# Autodesk Inventor assembly: base
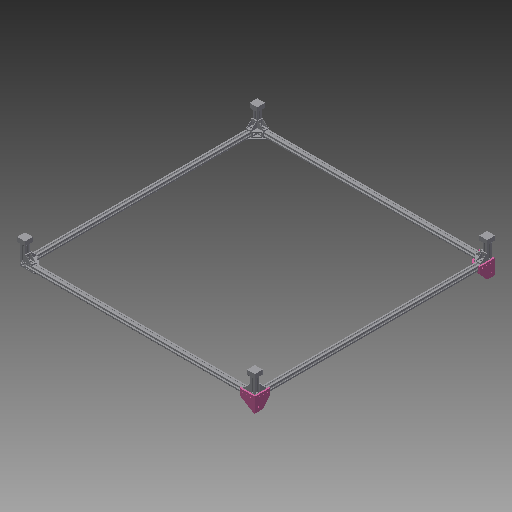
[picture p0: Inventor's stored thumbnail of the model, 512x512]
Saved by Autodesk Inventor 2019 (Build 230136000, 136)
## iProperties
Created: 2019-04-21
Part Number: base
Document SubType Name: Assembly
Designer: Alex Jones
Author: Alex Jones
## Documents named in this file (9)
- C:\Users\Alex Jones\Documents\Inventor\CNC\base.iam
- C:\Users\Alex Jones\Documents\Inventor\CNC\2020-1m.ipt
- C:\Users\Alex Jones\Documents\Inventor\CNC\2020-90.ipt
- C:\Users\Alex Jones\Documents\Inventor\CNC\2020-90-plate.ipt
- C:\Users\Alex Jones\Documents\Inventor\CNC\2020-3in.ipt
- C:\Users\Alex Jones\Documents\Inventor\CNC\baseFoot.ipt
- C:\Users\Alex Jones\Documents\Inventor\CNC\2020-950mm.ipt
- C:\Users\Alex Jones\Documents\Inventor\CNC\xIdler.ipt
- C:\Users\Alex Jones\Documents\Inventor\CNC\xIdlerMirror.ipt
## Components (28 placed, 8 different names)
1. 2020-950mm:1 — Mate:1, Flush:1, Flush:2, Flush:4, Mate:3, Flush:5, Flush:6, Flush:7, Flush:8, Flush:18, Mate:13, Mate:16, Flush:26, Mate:17, Flush:27, Mate:18, Flush:29, Mate:22, Mate:50
2. 2020-90:1 — Mate:1, Flush:1, Flush:2, Mate:2, Flush:3
3. 2020-1m:2 — Mate:4, Flush:7, Flush:8, Mate:5, Flush:10, Flush:12, Mate:12, Flush:19, Flush:20, Flush:21, Mate:14, Flush:28, Flush:30, Mate:21, Flush:35, Mate:31
4. 2020-1m:3 — Mate:2, Flush:3, Flush:4, Mate:6, Flush:9, Mate:9, Flush:23, Mate:15, Flush:25, Mate:24, Flush:32, Mate:45, Mate:46, Mate:47, Mate:49, Mate:51
5. 2020-950mm:2 — Mate:7, Flush:11, Mate:8, Mate:9, Flush:12, Flush:17, Flush:22, Flush:24, Flush:33, Mate:27, Mate:28, Flush:34, Mate:48
6. 2020-90:2 — Mate:6, Flush:9, Mate:8
7. 2020-90:3 — Mate:3, Flush:5, Flush:6, Mate:4
8. 2020-90:4 — Mate:5, Flush:10, Mate:7, Flush:11
9. 2020-90-plate:1 — Flush:18, Flush:19, Mate:13
10. 2020-90-plate:2 — Mate:12, Flush:17, Flush:20
11. 2020-3in:1 — Flush:21, Flush:22, Mate:14, Mate:29, Mate:30, Mate:35, Mate:36, Mate:37
12. 2020-3in:2 — Mate:17, Flush:27, Flush:28, Mate:19, Mate:20, Mate:38, Mate:39, Mate:40
13. 2020-3in:3 — Mate:16, Flush:25, Flush:26, Flush:31, Mate:23, Mate:25, Mate:41, Mate:42, Mate:43
14. 2020-3in:4 — Flush:23, Flush:24, Mate:15, Mate:26, Mate:32, Mate:33, Mate:34, Mate:44, Flush:36
15. 2020-90:5 — Mate:18, Flush:29, Mate:19
16. 2020-90:6 — Mate:20, Flush:30, Mate:21
17. 2020-90:7 — Mate:22, Flush:31, Mate:23
18. 2020-90:8 — Mate:24, Flush:32, Mate:25
19. 2020-90:9 — Flush:33, Mate:26, Mate:27
20. 2020-90:10 — Mate:28, Flush:34, Mate:29
21. 2020-90:11 — Flush:35, Mate:30, Mate:31
22. baseFoot:1 — Mate:32, Mate:33, Mate:34
23. baseFoot:2 — Mate:35, Mate:36, Mate:37
24. baseFoot:3 — Mate:38, Mate:39, Mate:40
25. baseFoot:4 — Mate:41, Mate:42, Mate:43
26. 2020-90:12 — Mate:44, Flush:36, Mate:45
27. xIdler:1 — Mate:46, Mate:47, Mate:48
28. xIdlerMirror:1 — Mate:49, Mate:50, Mate:51
## Relationships (81: Mate 49, Flush 32)
- Mate:1: 2020-950mm:1 ↔ 2020-90:1
- Flush:1: 2020-950mm:1 ↔ 2020-90:1
- Flush:2: 2020-950mm:1 ↔ 2020-90:1
- Mate:2: 2020-90:1 ↔ 2020-1m:3
- Flush:3: 2020-90:1 ↔ 2020-1m:3
- Flush:4: 2020-950mm:1 ↔ 2020-1m:3
- Mate:3: 2020-950mm:1 ↔ 2020-90:3
- Flush:5: 2020-950mm:1 ↔ 2020-90:3
- Flush:6: 2020-950mm:1 ↔ 2020-90:3
- Mate:4: 2020-1m:2 ↔ 2020-90:3
- Flush:7: 2020-950mm:1 ↔ 2020-1m:2
- Flush:8: 2020-950mm:1 ↔ 2020-1m:2
- Mate:5: 2020-1m:2 ↔ 2020-90:4
- Mate:6: 2020-1m:3 ↔ 2020-90:2
- Flush:9: 2020-1m:3 ↔ 2020-90:2
- Flush:10: 2020-1m:2 ↔ 2020-90:4
- Mate:7: 2020-950mm:2 ↔ 2020-90:4
- Flush:11: 2020-950mm:2 ↔ 2020-90:4
- Mate:8: 2020-950mm:2 ↔ 2020-90:2
- Mate:9: 2020-1m:3 ↔ 2020-950mm:2
- Flush:12: 2020-1m:2 ↔ 2020-950mm:2
- Mate:12: 2020-1m:2 ↔ 2020-90-plate:2
- Flush:17: 2020-950mm:2 ↔ 2020-90-plate:2
- Flush:18: 2020-950mm:1 ↔ 2020-90-plate:1
- Flush:19: 2020-1m:2 ↔ 2020-90-plate:1
- Mate:13: 2020-950mm:1 ↔ 2020-90-plate:1
- Flush:20: 2020-1m:2 ↔ 2020-90-plate:2
- Flush:21: 2020-1m:2 ↔ 2020-3in:1
- Flush:22: 2020-950mm:2 ↔ 2020-3in:1
- Mate:14: 2020-1m:2 ↔ 2020-3in:1
- Flush:23: 2020-1m:3 ↔ 2020-3in:4
- Flush:24: 2020-950mm:2 ↔ 2020-3in:4
- Mate:15: 2020-1m:3 ↔ 2020-3in:4
- Mate:16: 2020-950mm:1 ↔ 2020-3in:3
- Flush:25: 2020-1m:3 ↔ 2020-3in:3
- Flush:26: 2020-950mm:1 ↔ 2020-3in:3
- Mate:17: 2020-950mm:1 ↔ 2020-3in:2
- Flush:27: 2020-950mm:1 ↔ 2020-3in:2
- Flush:28: 2020-1m:2 ↔ 2020-3in:2
- Mate:18: 2020-950mm:1 ↔ 2020-90:5
- Flush:29: 2020-950mm:1 ↔ 2020-90:5
- Mate:19: 2020-3in:2 ↔ 2020-90:5
- Mate:20: 2020-3in:2 ↔ 2020-90:6
- Flush:30: 2020-1m:2 ↔ 2020-90:6
- Mate:21: 2020-1m:2 ↔ 2020-90:6
- Mate:22: 2020-950mm:1 ↔ 2020-90:7
- Flush:31: 2020-3in:3 ↔ 2020-90:7
- Mate:23: 2020-3in:3 ↔ 2020-90:7
- Mate:24: 2020-1m:3 ↔ 2020-90:8
- Flush:32: 2020-1m:3 ↔ 2020-90:8
- Mate:25: 2020-3in:3 ↔ 2020-90:8
- Flush:33: 2020-950mm:2 ↔ 2020-90:9
- Mate:26: 2020-3in:4 ↔ 2020-90:9
- Mate:27: 2020-950mm:2 ↔ 2020-90:9
- Mate:28: 2020-950mm:2 ↔ 2020-90:10
- Flush:34: 2020-950mm:2 ↔ 2020-90:10
- Mate:29: 2020-3in:1 ↔ 2020-90:10
- Flush:35: 2020-1m:2 ↔ 2020-90:11
- Mate:30: 2020-3in:1 ↔ 2020-90:11
- Mate:31: 2020-1m:2 ↔ 2020-90:11
- Mate:32: 2020-3in:4 ↔ baseFoot:1
- Mate:33: 2020-3in:4 ↔ baseFoot:1
- Mate:34: 2020-3in:4 ↔ baseFoot:1
- Mate:35: 2020-3in:1 ↔ baseFoot:2
- Mate:36: 2020-3in:1 ↔ baseFoot:2
- Mate:37: 2020-3in:1 ↔ baseFoot:2
- Mate:38: 2020-3in:2 ↔ baseFoot:3
- Mate:39: 2020-3in:2 ↔ baseFoot:3
- Mate:40: 2020-3in:2 ↔ baseFoot:3
- Mate:41: 2020-3in:3 ↔ baseFoot:4
- Mate:42: 2020-3in:3 ↔ baseFoot:4
- Mate:43: 2020-3in:3 ↔ baseFoot:4
- Mate:44: 2020-3in:4 ↔ 2020-90:12
- Flush:36: 2020-3in:4 ↔ 2020-90:12
- Mate:45: 2020-1m:3 ↔ 2020-90:12
- Mate:46: 2020-1m:3 ↔ xIdler:1
- Mate:47: 2020-1m:3 ↔ xIdler:1
- Mate:48: 2020-950mm:2 ↔ xIdler:1
- Mate:49: 2020-1m:3 ↔ xIdlerMirror:1
- Mate:50: 2020-950mm:1 ↔ xIdlerMirror:1
- Mate:51: 2020-1m:3 ↔ xIdlerMirror:1
